# Autodesk Inventor assembly: MGN12H Block
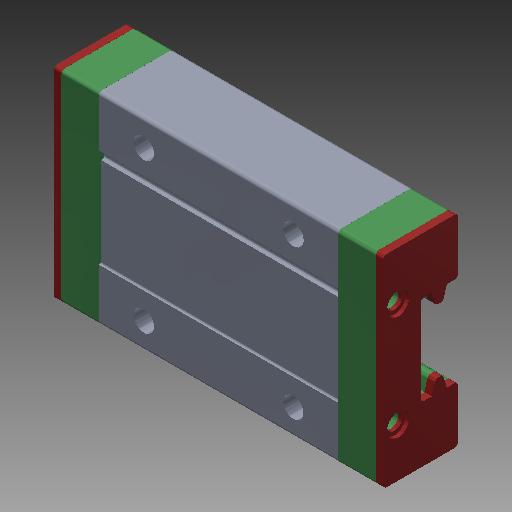
[picture p0: Inventor's stored thumbnail of the model, 512x512]
Saved by Autodesk Inventor 2019 (Build 230136000, 136)
## iProperties
Created: 2018-10-07
Part Number: MGN12H Block
Document SubType Name: Assembly
Designer: Ax
Mass: 8.35525 g
Surface Area: 68.7236 cm^2
Volume: 8.35525 cm^3
Density: 1 g/cm^3
Author: Ax
## Documents named in this file (4)
- C:\Users\Ax\Google Drive\Inventor\Library\mgn12-sliding-block-linear-guide-1.snapshot.2\MGN12H Block.iam
- C:\Users\Ax\Google Drive\Inventor\Library\mgn12-sliding-block-linear-guide-1.snapshot.2\Main Block.ipt
- C:\Users\Ax\Google Drive\Inventor\Library\mgn12-sliding-block-linear-guide-1.snapshot.2\Green End Cap.ipt
- C:\Users\Ax\Google Drive\Inventor\Library\mgn12-sliding-block-linear-guide-1.snapshot.2\Red End Cap.ipt
## Components (5 placed, 3 different names)
1. Main Block:1 — Mate:2, Mate:3, Mate:5, Mate:6, Mate:7, Mate:8
2. Green End Cap:1 — Mate:5, Mate:6, Mate:8, Mate:9, Mate:10, Mate:11
3. Red End Cap:1 — Mate:9, Mate:10, Mate:11
4. Green End Cap:2 — Mate:2, Mate:3, Mate:7, Mate:12, Mate:13, Mate:14
5. Red End Cap:2 — Mate:12, Mate:13, Mate:14
## Relationships (12: Mate 12)
- Mate:2: Main Block:1 ↔ Green End Cap:2
- Mate:3: Main Block:1 ↔ Green End Cap:2
- Mate:5: Main Block:1 ↔ Green End Cap:1
- Mate:6: Main Block:1 ↔ Green End Cap:1
- Mate:7: Main Block:1 ↔ Green End Cap:2
- Mate:8: Main Block:1 ↔ Green End Cap:1
- Mate:9: Green End Cap:1 ↔ Red End Cap:1
- Mate:10: Green End Cap:1 ↔ Red End Cap:1
- Mate:11: Green End Cap:1 ↔ Red End Cap:1
- Mate:12: Green End Cap:2 ↔ Red End Cap:2
- Mate:13: Green End Cap:2 ↔ Red End Cap:2
- Mate:14: Green End Cap:2 ↔ Red End Cap:2
